# Autodesk Inventor assembly: POM_T5_05
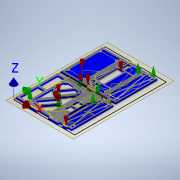
[picture p0: Inventor's stored thumbnail of the model, 180x180]
Saved by Autodesk Inventor 2022.3 (Build 263350000, 350)
## iProperties
Created: 2022-09-28
Part Number: POM_T5_05
Document SubType Name: Assembly
Designer: Masato
Author: Masato
## Documents named in this file (8)
- C:\Users\Masato\Documents\Inventor\Inventor for CIT Brains\SUSTAINA-OP - Cockpit mate\Cam\POM_T5\POM_T5_05.iam
- C:\Users\Masato\Documents\Inventor\Inventor for CIT Brains\SUSTAINA-OP - Cockpit mate\Cam\DisposableBoard.ipt
- C:\Users\Masato\Documents\Inventor\Inventor for CIT Brains\SUSTAINA-OP - Cockpit mate\UpperBody\Cockpit\Cockpit_back_frame.ipt
- C:\Users\Masato\Documents\Inventor\Inventor for CIT Brains\SUSTAINA-OP - Cockpit mate\UpperBody\Cockpit\Cockpit_battery_frame.ipt
- C:\Users\Masato\Documents\Inventor\Inventor for CIT Brains\SUSTAINA-OP - Cockpit mate\UpperBody\Cockpit\Cockpit_carrier_board_frame.ipt
- C:\Users\Masato\Documents\Inventor\Inventor for CIT Brains\SUSTAINA-OP - Cockpit mate\UpperBody\Cockpit\Cockpit_circuit_board_frame.ipt
- C:\Users\Masato\Documents\Inventor\Inventor for CIT Brains\SUSTAINA-OP - Cockpit mate\UpperBody\Cockpit\Cockpit_front_frame.ipt
- C:\Users\Masato\Documents\Inventor\Inventor for CIT Brains\SUSTAINA-OP - Cockpit mate\UpperBody\Cockpit\Cockpit_top_frame.ipt
## Components (9 placed, 7 different names)
1. DisposableBoard:1 — フラッシュ:1, フラッシュ:2, フラッシュ:3, フラッシュ:4, フラッシュ:5, フラッシュ:8
2. Cockpit_back_frame:1 — メイト:5, メイト:14, フラッシュ:10, フラッシュ:11, メイト:15, メイト:16
3. Cockpit_battery_frame:1 — メイト:4, フラッシュ:7, メイト:13
4. Cockpit_carrier_board_frame:1 — メイト:17, 正接:3, 正接:4, メイト:19
5. Cockpit_circuit_board_frame:1 — メイト:2, フラッシュ:5, フラッシュ:6, フラッシュ:8, メイト:12, フラッシュ:9, メイト:14, 正接:1, 正接:2, メイト:18, 正接:3, 正接:4, メイト:19
6. Cockpit_front_frame:1 — メイト:1, フラッシュ:9, フラッシュ:10, メイト:15
7. Cockpit_top_frame:1 — メイト:8, フラッシュ:6, フラッシュ:7, メイト:12, メイト:13
8. Cockpit_carrier_board_frame:2 — メイト:10, 正接:1, 正接:2, メイト:18
9. Cockpit_battery_frame:2 — メイト:6, フラッシュ:11, メイト:16
## Relationships (30: Mate 15, Flush 11, Tangent 4)
- フラッシュ:1 [Flush]: DisposableBoard:1
- フラッシュ:2 [Flush]: DisposableBoard:1
- フラッシュ:3 [Flush]: DisposableBoard:1
- フラッシュ:4 [Flush]: DisposableBoard:1
- メイト:1 [Mate]: Cockpit_front_frame:1
- メイト:2 [Mate]: Cockpit_circuit_board_frame:1
- メイト:4 [Mate]: Cockpit_battery_frame:1
- メイト:5 [Mate]: Cockpit_back_frame:1
- メイト:6 [Mate]: Cockpit_battery_frame:2
- メイト:8 [Mate]: Cockpit_top_frame:1
- メイト:10 [Mate]: Cockpit_carrier_board_frame:2
- フラッシュ:5 [Flush] (-2 mm): DisposableBoard:1 ↔ Cockpit_circuit_board_frame:1
- フラッシュ:6 [Flush]: Cockpit_circuit_board_frame:1 ↔ Cockpit_top_frame:1
- フラッシュ:7 [Flush]: Cockpit_battery_frame:1 ↔ Cockpit_top_frame:1
- フラッシュ:8 [Flush] (-2 mm): DisposableBoard:1 ↔ Cockpit_circuit_board_frame:1
- メイト:12 [Mate] (2.1 mm): Cockpit_circuit_board_frame:1 ↔ Cockpit_top_frame:1
- メイト:13 [Mate] (2.1 mm): Cockpit_battery_frame:1 ↔ Cockpit_top_frame:1
- フラッシュ:9 [Flush]: Cockpit_circuit_board_frame:1 ↔ Cockpit_front_frame:1
- メイト:14 [Mate] (2.1 mm): Cockpit_back_frame:1 ↔ Cockpit_circuit_board_frame:1
- フラッシュ:10 [Flush]: Cockpit_back_frame:1 ↔ Cockpit_front_frame:1
- フラッシュ:11 [Flush]: Cockpit_back_frame:1 ↔ Cockpit_battery_frame:2
- メイト:15 [Mate] (2.1 mm): Cockpit_back_frame:1 ↔ Cockpit_front_frame:1
- メイト:16 [Mate] (2.1 mm): Cockpit_back_frame:1 ↔ Cockpit_battery_frame:2
- メイト:17 [Mate]: Cockpit_carrier_board_frame:1
- 正接:1 [Tangent] (2.1 mm): Cockpit_circuit_board_frame:1 ↔ Cockpit_carrier_board_frame:2
- 正接:2 [Tangent] (2.1 mm): Cockpit_circuit_board_frame:1 ↔ Cockpit_carrier_board_frame:2
- メイト:18 [Mate] (2.1 mm): Cockpit_circuit_board_frame:1 ↔ Cockpit_carrier_board_frame:2
- 正接:3 [Tangent] (2.1 mm): Cockpit_carrier_board_frame:1 ↔ Cockpit_circuit_board_frame:1
- 正接:4 [Tangent] (2.1 mm): Cockpit_carrier_board_frame:1 ↔ Cockpit_circuit_board_frame:1
- メイト:19 [Mate] (2.1 mm): Cockpit_carrier_board_frame:1 ↔ Cockpit_circuit_board_frame:1
